# Autodesk Inventor assembly: 17HS4401S Stepper Motor
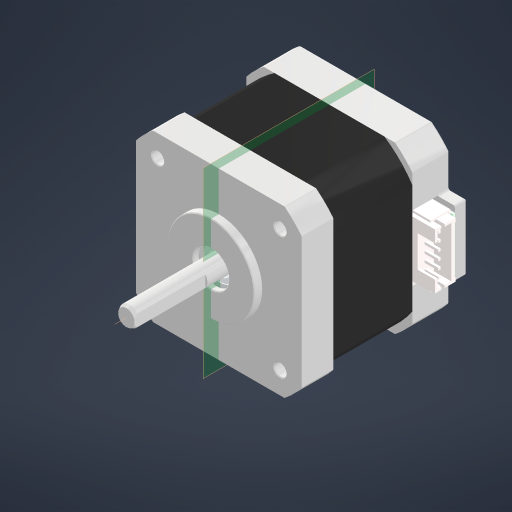
[picture p0: Inventor's stored thumbnail of the model, 512x512]
Saved by Autodesk Inventor 2024 (Build 280153000, 153)
## iProperties
Created: 2024-09-10
Part Number: 17HS4401S Stepper Motor
Description: FreeCAD Model
Document SubType Name: Assembly
Designer: schar
Authority: Unknown
Mass: 271 g
Surface Area: 223.527 cm^2
Volume: 62.5855 cm^3
Sending System: FreeCAD
Preprocessor: Open CASCADE STEP processor 7.6
Title: Open CASCADE Shape Model
## Documents named in this file (9)
- C:\Users\schar\Desktop\FloatingFace\models\17HS4401S_Stepper_Motor\17HS4401S_Stepper_Motor.iam
- C:\Users\schar\Desktop\FloatingFace\models\17HS4401S_Stepper_Motor\rear end cap.ipt
- C:\Users\schar\Desktop\FloatingFace\models\17HS4401S_Stepper_Motor\rear bearing.ipt
- C:\Users\schar\Desktop\FloatingFace\models\17HS4401S_Stepper_Motor\connector.ipt
- C:\Users\schar\Desktop\FloatingFace\models\17HS4401S_Stepper_Motor\shaft.ipt
- C:\Users\schar\Desktop\FloatingFace\models\17HS4401S_Stepper_Motor\stator.ipt
- C:\Users\schar\Desktop\FloatingFace\models\17HS4401S_Stepper_Motor\front end cap.ipt
- C:\Users\schar\Desktop\FloatingFace\models\17HS4401S_Stepper_Motor\front bearing.ipt
- C:\Users\schar\Desktop\FloatingFace\models\17HS4401S_Stepper_Motor\M3x10-Screw.ipt
## Components (11 placed, 11 different names)
1. 1 — Symmetry:1
2. 2
3. 3
4. 4 — Mate:1
5. 5
6. 6 — Symmetry:1
7. 7
8. 8
9. 9
10. 10
11. 11
## Relationships (2: Mate 1, Symmetry 1)
- Mate:1: 4
- Symmetry:1: 1 ↔ 6
